# Autodesk Inventor assembly: final assembly
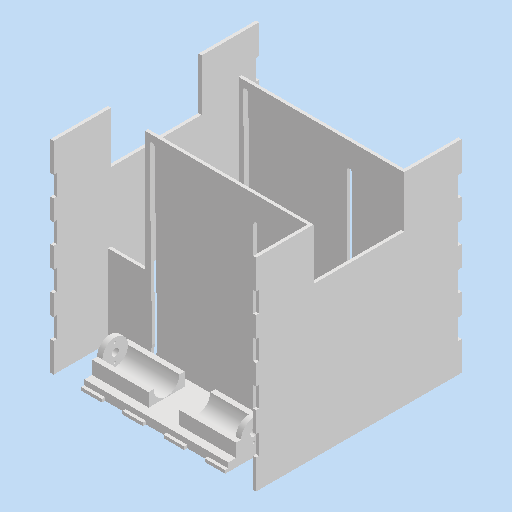
[picture p0: Inventor's stored thumbnail of the model, 512x512]
Saved by Autodesk Inventor 2026 (Build 300175000, 175)
## iProperties
Created: 2026-02-10
Part Number: final assembly
Document SubType Name: Assembly
Designer: mones
Author: mones
## Documents named in this file (6)
- C:\Users\mones\OneDrive - Northeastern University\unibots\Unibots_NULondon\hardware\final assembly\final assembly.iam
- C:\Users\mones\OneDrive - Northeastern University\unibots\Unibots_NULondon\hardware\chassis\final\inside walls left.ipt
- C:\Users\mones\OneDrive - Northeastern University\unibots\Unibots_NULondon\hardware\chassis\final\inside walls right.ipt
- C:\Users\mones\OneDrive - Northeastern University\unibots\Unibots_NULondon\hardware\motor_mounts\bottom plate left\bottom plate.ipt
- C:\Users\mones\OneDrive - Northeastern University\unibots\Unibots_NULondon\hardware\chassis\final\back plate.ipt
- C:\Users\mones\OneDrive - Northeastern University\unibots\Unibots_NULondon\hardware\chassis\final\front plate.ipt
## Components (6 placed, 5 different names)
1. inside walls left:1 — Mate:1, Mate:2, Mate:8, Mate:9, Mate:10
2. inside walls right:1 — Mate:3, Mate:4, Mate:5, Mate:6, Mate:7
3. bottom plate:1 — Mate:3, Mate:4
4. bottom plate:2 — Mate:1, Mate:2
5. back plate:1 — Mate:5, Mate:6, Mate:7, Mate:8
6. front plate:1 — Mate:9, Mate:10
## Relationships (10: Mate 10)
- Mate:1: inside walls left:1 ↔ bottom plate:2
- Mate:2: inside walls left:1 ↔ bottom plate:2
- Mate:3: inside walls right:1 ↔ bottom plate:1
- Mate:4: inside walls right:1 ↔ bottom plate:1
- Mate:5: inside walls right:1 ↔ back plate:1
- Mate:6: inside walls right:1 ↔ back plate:1
- Mate:7: inside walls right:1 ↔ back plate:1
- Mate:8: inside walls left:1 ↔ back plate:1
- Mate:9: inside walls left:1 ↔ front plate:1
- Mate:10: inside walls left:1 ↔ front plate:1
